# Autodesk Inventor assembly: Frezowanie No.2
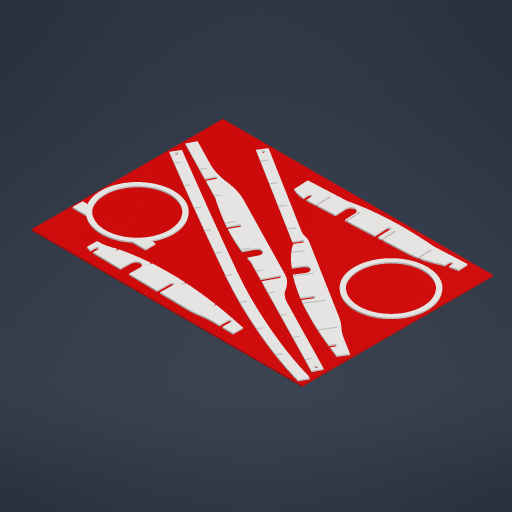
[picture p0: Inventor's stored thumbnail of the model, 512x512]
Saved by Autodesk Inventor 2023 (Build 270158000, 158)
## iProperties
Created: 2023-04-06
Part Number: Frezowanie No.2
Document SubType Name: Assembly
Designer: szykr
Author: szykr
## Documents named in this file (9)
- D:\Folder Instalacyjny\GitHub Pliki\Solaris\new model\Frez\Frezowanie No.2.iam
- D:\Folder Instalacyjny\GitHub Pliki\Solaris\new model\Frez\Laminat297x210.ipt
- D:\Folder Instalacyjny\GitHub Pliki\Solaris\new model\Frez\Dlugie party(32-47)\Solid40.ipt
- D:\Folder Instalacyjny\GitHub Pliki\Solaris\new model\Frez\Dlugie party(32-47)\Solid44.ipt
- D:\Folder Instalacyjny\GitHub Pliki\Solaris\new model\Frez\Dlugie party(32-47)\Solid46.ipt
- D:\Folder Instalacyjny\GitHub Pliki\Solaris\new model\Frez\Troche Mniejsze(2-31)\Solid5.ipt
- D:\Folder Instalacyjny\GitHub Pliki\Solaris\new model\Frez\Troche Mniejsze(2-31)\Solid15.ipt
- D:\Folder Instalacyjny\GitHub Pliki\Solaris\new model\Frez\Troche Mniejsze(2-31)\Solid29.ipt
- D:\Folder Instalacyjny\GitHub Pliki\Solaris\new model\Frez\Troche Mniejsze(2-31)\Solid30.ipt
## Components (8 placed, 8 different names)
1. Laminat297x210:1 — Angle:1, Mate:1, Mate:2, Mate:3, Mate:4, Mate:5, Mate:6, Mate:7
2. Solid40:1 — Angle:1, Mate:1
3. Solid44:1 — Mate:2
4. Solid46:1 — Mate:3
5. Solid5:1 — Mate:4
6. Solid15:1 — Mate:5
7. Solid29:1 — Mate:6
8. Solid30:1 — Mate:7
## Relationships (8: Mate 7, Angle 1)
- Angle:1 (0 deg): Laminat297x210:1 ↔ Solid40:1
- Mate:1: Laminat297x210:1 ↔ Solid40:1
- Mate:2: Laminat297x210:1 ↔ Solid44:1
- Mate:3: Laminat297x210:1 ↔ Solid46:1
- Mate:4: Laminat297x210:1 ↔ Solid5:1
- Mate:5: Laminat297x210:1 ↔ Solid15:1
- Mate:6: Laminat297x210:1 ↔ Solid29:1
- Mate:7: Laminat297x210:1 ↔ Solid30:1
